# Autodesk Inventor assembly: SAR330 x 2 + regular couplers left offset
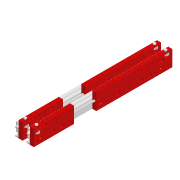
[picture p0: Inventor's stored thumbnail of the model, 180x180]
Saved by Autodesk Inventor 2020 (Build 240168000, 168)
## iProperties
Created: 2019-11-17
Part Number: SAR330 x 2 + regular couplers left offset
Document SubType Name: Assembly
Designer: ball
Author: ball
## Documents named in this file (2)
- C:\FTC\FTC8863CAD\2019 Robot\Delivery\SAR330 x 2 + regular couplers left offset.iam
- C:\FTC\FTC8863CAD\2019 Robot\Delivery\SAR330 + regular couplers left offset.iam
## Components (2 placed, 1 different names)
1. SAR330 + regular couplers left offset:2 [sub-assembly]
2. SAR330 + regular couplers left offset:1 [sub-assembly]
## Relationships (3: Mate 3)
- [Mate]: SAR330 + regular couplers left offset:2 ↔ SAR330 + regular couplers left offset:1
- [Mate]: SAR330 + regular couplers left offset:2 ↔ SAR330 + regular couplers left offset:1
- [Mate]: SAR330 + regular couplers left offset:2 ↔ SAR330 + regular couplers left offset:1
